# Autodesk Inventor assembly: левая лапа - сборка
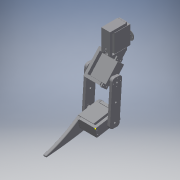
[picture p0: Inventor's stored thumbnail of the model, 180x180]
Saved by Autodesk Inventor 2019 (Build 230136000, 136)
## iProperties
Created: 2019-09-06
Part Number: левая лапа - сборка
Material: Типовые
Document SubType Name: Assembly
Designer: Iliga
Author: Iliga
## Documents named in this file (7)
- C:\Users\Iliga\Desktop\робот\левая лапа - сборка.iam
- C:\Users\Iliga\Desktop\робот\двигатель.ipt
- C:\Users\Iliga\Desktop\робот\Юля\kreplenie3.ipt
- C:\Users\Iliga\Desktop\робот\Юля\kreplenie1.ipt
- C:\Users\Iliga\Desktop\робот\Юля\peregorodka.ipt
- C:\Users\Iliga\Desktop\робот\Юля\ship.ipt
- C:\Users\Iliga\Desktop\робот\Юля\kreplenie2.ipt
## Components (9 placed, 6 different names)
1. двигатель:1 — Совмещение:2, Совмещение:26, Совмещение:27
2. kreplenie3:1 — Совмещение:2, Совмещение:3, Заподлицо:2, Заподлицо:3, Совмещение:24, Совмещение:26, Совмещение:27
3. kreplenie1:1 — Совмещение:3, Заподлицо:2, Заподлицо:3, Совмещение:4, Совмещение:6, Совмещение:7, Совмещение:21
4. двигатель:2 — Совмещение:4, Совмещение:8, Совмещение:9, Совмещение:21, Совмещение:24
5. peregorodka:1 — Совмещение:6, Совмещение:7, Совмещение:22, Совмещение:25
6. peregorodka:2 — Совмещение:8, Совмещение:9, Совмещение:18, Совмещение:22
7. ship:1 — Совмещение:11, Совмещение:12, Совмещение:16
8. двигатель:3 — Совмещение:11, Совмещение:12, Совмещение:15, Заподлицо:5, Совмещение:16, Совмещение:17, Совмещение:25
9. kreplenie2:1 — Совмещение:15, Заподлицо:5, Совмещение:17, Совмещение:18
## Relationships (22: Mate 19, Flush 3)
- Совмещение:2 [Mate]: двигатель:1 ↔ kreplenie3:1
- Совмещение:3 [Mate]: kreplenie3:1 ↔ kreplenie1:1
- Заподлицо:2 [Flush]: kreplenie3:1 ↔ kreplenie1:1
- Заподлицо:3 [Flush]: kreplenie3:1 ↔ kreplenie1:1
- Совмещение:4 [Mate]: kreplenie1:1 ↔ двигатель:2
- Совмещение:6 [Mate]: kreplenie1:1 ↔ peregorodka:1
- Совмещение:7 [Mate]: kreplenie1:1 ↔ peregorodka:1
- Совмещение:8 [Mate]: двигатель:2 ↔ peregorodka:2
- Совмещение:9 [Mate]: двигатель:2 ↔ peregorodka:2
- Совмещение:11 [Mate]: ship:1 ↔ двигатель:3
- Совмещение:12 [Mate]: ship:1 ↔ двигатель:3
- Совмещение:15 [Mate]: двигатель:3 ↔ kreplenie2:1
- Заподлицо:5 [Flush]: двигатель:3 ↔ kreplenie2:1
- Совмещение:16 [Mate]: ship:1 ↔ двигатель:3
- Совмещение:17 [Mate]: двигатель:3 ↔ kreplenie2:1
- Совмещение:18 [Mate]: peregorodka:2 ↔ kreplenie2:1
- Совмещение:21 [Mate]: kreplenie1:1 ↔ двигатель:2
- Совмещение:22 [Mate]: peregorodka:1 ↔ peregorodka:2
- Совмещение:24 [Mate]: kreplenie3:1 ↔ двигатель:2
- Совмещение:25 [Mate]: peregorodka:1 ↔ двигатель:3
- Совмещение:26 [Mate]: двигатель:1 ↔ kreplenie3:1
- Совмещение:27 [Mate]: двигатель:1 ↔ kreplenie3:1
